# Autodesk Inventor assembly: sm_connection
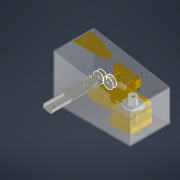
[picture p0: Inventor's stored thumbnail of the model, 180x180]
Saved by Autodesk Inventor 2021 (Build 250183000, 183)
## iProperties
Created: 2021-06-22
Part Number: sm_connection
Document SubType Name: Assembly
Designer: Watchdog
Mass: 4766.5 g
Surface Area: 4999.63 cm^2
Volume: 1578.22 cm^3
Density: 3.02017 g/cm^3
Author: Watchdog
## Documents named in this file (9)
- C:\Users\Watchdog\OneDrive - Flinders\Advn Mech Design Shared\6_Development\2_Design\inventor\securing_mechanism\connection\sm_connection.iam
- C:\Users\Watchdog\OneDrive - Flinders\Advn Mech Design Shared\6_Development\2_Design\inventor\securing_mechanism\connection\gear_khk_SUS1-28J10.ipt
- C:\Users\Watchdog\OneDrive - Flinders\Advn Mech Design Shared\6_Development\2_Design\inventor\securing_mechanism\connection\member_s2c.ipt
- C:\Users\Watchdog\OneDrive - Flinders\Advn Mech Design Shared\6_Development\2_Design\inventor\support\reel\motor.ipt
- C:\Users\Watchdog\OneDrive - Flinders\Advn Mech Design Shared\6_Development\2_Design\inventor\securing_mechanism\connection\box.ipt
- C:\Users\Watchdog\OneDrive - Flinders\Advn Mech Design Shared\6_Development\2_Design\inventor\securing_mechanism\connection\secureingReel.ipt
- C:\Users\Watchdog\OneDrive - Flinders\Advn Mech Design Shared\6_Development\2_Design\inventor\securing_mechanism\connection\bearingSeat.ipt
- C:\Users\Watchdog\OneDrive - Flinders\Advn Mech Design Shared\6_Development\2_Design\inventor\securing_mechanism\connection\SKF_16100.iam
- C:\Users\Watchdog\OneDrive - Flinders\Advn Mech Design Shared\6_Development\2_Design\inventor\params.xlsx
## Components (9 placed, 7 different names)
1. gear_khk_SUS1-28J10:1 — Mate:22, Mate:23
2. member_s2c:1 — Mate:2, Mate:6, Mate:19, Mate:20, Mate:22, Mate:23, Angle:6
3. motor:1 — Angle:3, Mate:10, Mate:25, Angle:5, Flush:2, Mate:26
4. gear_khk_SUS1-28J10:2 — Mate:25, Angle:5, Flush:2
5. motor:2 — Angle:3, Mate:11, Mate:12, Mate:13, Mate:14, Angle:4, Mate:15
6. box:1 — Mate:6, Mate:10, Mate:11, Mate:12, Mate:13, Mate:17, Mate:21, Mate:24, Mate:26, Flush:3, Flush:4
7. secureingReel:1 — Mate:14, Angle:4, Mate:15
8. bearingSeat:1 — Mate:17, Mate:21
9. SKF_16100:1 [sub-assembly] — Mate:19, Mate:20, Mate:24
## Relationships (24: Mate 17, Angle 4, Flush 3)
- Mate:2: member_s2c:1
- Mate:6: member_s2c:1 ↔ box:1
- Angle:3 (0 deg): motor:1 ↔ motor:2
- Mate:10: motor:1 ↔ box:1
- Mate:11: motor:2 ↔ box:1
- Mate:12: motor:2 ↔ box:1
- Mate:13: motor:2 ↔ box:1
- Mate:14: motor:2 ↔ secureingReel:1
- Angle:4 (180 deg): motor:2 ↔ secureingReel:1
- Mate:15: motor:2 ↔ secureingReel:1
- Mate:17: box:1 ↔ bearingSeat:1
- Mate:19: member_s2c:1 ↔ SKF_16100:1
- Mate:20: member_s2c:1 ↔ SKF_16100:1
- Mate:21: box:1 ↔ bearingSeat:1
- Mate:22: gear_khk_SUS1-28J10:1 ↔ member_s2c:1
- Mate:23: gear_khk_SUS1-28J10:1 ↔ member_s2c:1
- Mate:24: box:1 ↔ SKF_16100:1
- Mate:25: motor:1 ↔ gear_khk_SUS1-28J10:2
- Angle:5 (180 deg): motor:1 ↔ gear_khk_SUS1-28J10:2
- Flush:2: motor:1 ↔ gear_khk_SUS1-28J10:2
- Mate:26: motor:1 ↔ box:1
- Flush:3: box:1
- Flush:4: box:1
- Angle:6 (100 deg): member_s2c:1
## Named parameters: wheelchatir_pos_store_angle_0 = 90 deg, cover_base_thickness = 10 mm, cover_height_main = 900 mm, cover_length_main = 2200 mm, cover_mountHole_diameter = 10 mm, cover_mountHole_xSpacing = 900 mm, cover_mountHole_ySpacing = 550 mm, cover_shell_thickness = 10 mm, cover_side_openSize = 1400 mm, cover_side_thickness = 20 mm, cover_width_main = 1600 mm, hoop_angle_z = 45 deg, hoop_bearing_length = 5 deg, hoop_bushing12_od = 43 mm, hoop_bushing12_radialInterference = 0 mm, hoop_bushing12_thickness = 9.3 mm, hoop_bushing23_od = 27.3 mm, hoop_bushing23_radialInterference = 0 mm, hoop_bushing23_thickness = 1.9 mm, hoop_cable_diam = 5 mm, hoop_cable_pulley_diam = 22 mm, hoop_height_large = 450 mm, hoop_height_medium = 450 mm, hoop_height_small = 600 mm, hoop_length_large = 200 mm, hoop_length_medium = 700 mm, hoop_length_small = 700 mm, hoop_offset_x = 660 mm, hoop_radius_large = 3300 mm, hoop_tabs_hole = 12 mm, hoop_tabs_thickness = 6 mm, hoop_tabs_width = 50 mm, hoop_thickness_large = 4 mm, hoop_thickness_medium = 3.2 mm, hoop_thickness_small = 2 mm, hoop_width_large = 51 mm, hoop_width_medium = 33.7 mm, hoop_width_small = 25.4 mm, rack_tooth_addendum = 5 mm, rack_tooth_dedendum = 5 mm, rack_tooth_face_widh = 10 mm, rack_tooth_thickness = 5 mm, secure_arm_angle = 35 deg, secure_arm_hold_length = 50 mm, secure_arm_hold_thickness = 30 mm, secure_arm_length = 300 mm, secure_arm_radii = 9 mm, secure_arm_thickness = 30 mm, sm_varx_member_tolerance = 0 mm, sm_varx_pinPlate_aspectRatio = 2, sm_varx_pinPlate_holeDiameter = 5 mm, sm_varx_pinPlate_thickness = 5 mm, sm_varx_squareBarDimension = 30 mm, sm_varx_squareBarThickness = 2.5 mm, sm_varx_x = 100 mm, sm_varx_x_arms = 50 mm, sm_varx_y = 250 mm, sm_varx_z = 160 mm, support_baseClamp_lengthBuffer = 40 mm, support_baseClamp_platformLengthBuffer = 35 mm, support_baseClamp_platformThickness = 15 mm, support_baseClamp_platformWidthBuffer = 0 mm, support_baseClamp_sleeve_hole1Height = 50 mm, support_baseClamp_sleeve_hole2Height = 100 mm, support_baseClamp_sleeveHoleDiameter = 12 mm, support_baseClamp_sleeveSweepTerminationAngle = 55 deg, support_baseClamp_sleeveThickness = 20 mm, support_baseClamp_thickness = 8 mm, support_frame_clampHoleDiameter = 10 mm, support_frame_clampHoleSpacing = 100 mm, support_frame_endHoleBuffer = 45 mm, support_frame_length = 500 mm, support_frame_squareBarDimension = 50 mm, support_frame_squareBarFillet = 2 mm, support_frame_squareBarThickness = 5 mm, testHeight = 1000 mm, testLength = 1700 mm, testWidth = 1500 mm, wheelchair_deployed_height = 914 mm, wheelchair_deployed_length = 1067 mm, wheelchair_deployed_width = 635 mm, wheelchair_folded_width = 280 mm, wheelchair_wheel_radius = 240 mm, wheelchatir_pos_deploy_angle_0 = 65 deg, wheelchatir_pos_deploy_angle_1 = 20 deg, wheelchatir_pos_store_angle_1 = 20 deg
